# Autodesk Inventor assembly: extraTallPin
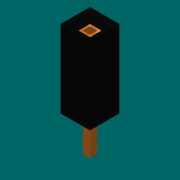
[picture p0: Inventor's stored thumbnail of the model, 180x180]
Saved by Autodesk Inventor 2016 SP1 (Build 200210100, 210)
## iProperties
Created: 2016-04-06
Part Number: extraTallPin
Document SubType Name: Assembly
Designer: sawai
Author: sawai
## Documents named in this file (3)
- C:\Users\sawai\OneDrive\projects\mppcInterface\cad\connector\2.54Header\female\1x1female.iam
- C:\Users\sawai\OneDrive\projects\mppcInterface\cad\connector\2.54Header\female\pinShroud.ipt
- C:\Users\sawai\OneDrive\projects\mppcInterface\cad\connector\2.54Header\female\pin.ipt
## Components (2 placed, 2 different names)
1. pinShroud:1 — Mate:1, Mate:2, Mate:3
2. pin:1 — Mate:1, Mate:2, Mate:3
## Relationships (3: Mate 3)
- Mate:1: pinShroud:1 ↔ pin:1
- Mate:2: pinShroud:1 ↔ pin:1
- Mate:3: pinShroud:1 ↔ pin:1
